# Autodesk Inventor assembly: link9_SubAssembly.ipt
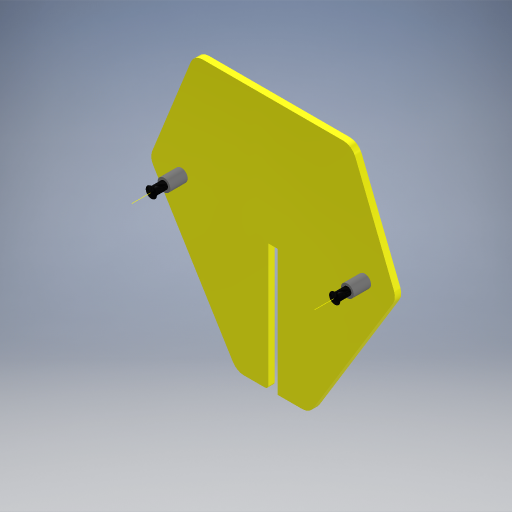
[picture p0: Inventor's stored thumbnail of the model, 512x512]
Saved by Autodesk Inventor 2024.1 (Build 281209000, 209)
## iProperties
Created: 2023-11-11
Part Number: link9_SubAssembly.ipt
Document SubType Name: Assembly
Designer: Camilo
Mass: 9.00832 g
Surface Area: 38.2093 cm^2
Volume: 3.33642 cm^3
Density: 2.7 g/cm^3
Author: Camilo
## Documents named in this file (4)
- D:\Documentos\MEGA\Universidad\2023-2\DinamicaComputacionalDeSistemasMulticuerpo\DinamicaComputacionalSistemasMulticuerpo\Proyecto\CAD\3D\link1_SubAssembly.iam
- D:\Documentos\MEGA\Universidad\2023-2\DinamicaComputacionalDeSistemasMulticuerpo\DinamicaComputacionalSistemasMulticuerpo\Proyecto\CAD\3D\link1.ipt
- D:\Documentos\MEGA\Universidad\2023-2\DinamicaComputacionalDeSistemasMulticuerpo\DinamicaComputacionalSistemasMulticuerpo\Proyecto\CAD\3D\spacer.ipt
- D:\Documentos\MEGA\Universidad\2023-2\DinamicaComputacionalDeSistemasMulticuerpo\DinamicaComputacionalSistemasMulticuerpo\Proyecto\CAD\3D\fix_bolt.ipt
## Components (5 placed, 3 different names)
1. link1:1 — Insert:1, Insert:2, Insert:3, Insert:4
2. spacer:1 — Insert:1
3. spacer:2 — Insert:2
4. fix_bolt:1 — Insert:3
5. fix_bolt:2 — Insert:4
## Relationships (4: Insert 4)
- Insert:1: link1:1 ↔ spacer:1
- Insert:2: link1:1 ↔ spacer:2
- Insert:3: link1:1 ↔ fix_bolt:1
- Insert:4: link1:1 ↔ fix_bolt:2
